# Autodesk Inventor assembly: one side of tower_MIR
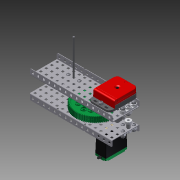
[picture p0: Inventor's stored thumbnail of the model, 180x180]
Saved by Autodesk Inventor 2014 SP1 (Build 180222100, 222)
## iProperties
Created: 2014-02-23
Part Number: one side of tower_MIR
Document SubType Name: Assembly
Designer: Ryan
Author: Ryan
## Documents named in this file (22)
- C:\Users\Ryan\Desktop\sw\toss up 4th robot\tower\one side of tower_MIR.iam
- C:\Users\Ryan\Desktop\sw\lib\Aperture VEX CAD Library\Metal\C Channel\5 x 15.ipt
- C:\Users\Ryan\Desktop\sw\lib\Aperture VEX CAD Library\Bearing Blocks\Bearing Block.ipt
- C:\Users\Ryan\Desktop\sw\lib\Aperture VEX CAD Library\Hardware\8-32\8-32 nylock.ipt
- C:\Users\Ryan\Desktop\sw\lib\Aperture VEX CAD Library\Hardware\8-32\8-32_.500.ipt
- C:\Users\Ryan\Desktop\sw\lib\Aperture VEX CAD Library\Spacers\thin\SPACER-0320-0125.ipt
- C:\Users\Ryan\Desktop\sw\lib\Aperture VEX CAD Library\Gears\High Strength Gears\HS-GEAR-12TOOTH.ipt
- C:\Users\Ryan\Desktop\sw\lib\Aperture VEX CAD Library\Hardware\8-32\8-32 nylock_MIR9.ipt
- C:\Users\Ryan\Desktop\sw\lib\Aperture VEX CAD Library\Spacers\thin\SPACER-0320-0500.ipt
- C:\Users\Ryan\Desktop\sw\lib\Aperture VEX CAD Library\Gears\High Strength Gears\Green HS 84.iam
- C:\Users\Ryan\Desktop\sw\lib\Aperture VEX CAD Library\Spacers\thin\SPACER-0320-0375.ipt
- C:\Users\Ryan\Desktop\sw\lib\Aperture VEX CAD Library\Hardware\Shaft Collar.ipt
- C:\Users\Ryan\Desktop\sw\lib\Aperture VEX CAD Library\Spacers\thin\SPACER-0320-0250.ipt
- C:\Users\Ryan\Desktop\sw\lib\Aperture VEX CAD Library\Standoffs\BEAM-1000.ipt
- C:\Users\Ryan\Desktop\sw\lib\Aperture VEX CAD Library\Hardware\8-32\8-32_.375.ipt
- C:\Users\Ryan\Desktop\sw\lib\Aperture VEX CAD Library\Standoffs\BEAM-0500.ipt
- C:\Users\Ryan\Desktop\sw\lib\Super Sonic Sparks VEX CAD Library\Motors & Sensors\2-Wire Motor 393-Without Wire.iam
- C:\Users\Ryan\Desktop\sw\lib\Aperture VEX CAD Library\Spacers\SPACER-0500-0250.ipt
- C:\Users\Ryan\Desktop\sw\lib\Aperture VEX CAD Library\Spacers\SPACER-0500-0625.ipt
- C:\Users\Ryan\Desktop\sw\lib\Aperture VEX CAD Library\Spacers\SPACER-0500-0125.ipt
- C:\Users\Ryan\Desktop\sw\lib\Aperture VEX CAD Library\Shaft\5.5 inch shaft.ipt
- C:\Users\Ryan\Desktop\sw\toss up 4th robot\tower\arm encoder.iam
## Components (66 placed, 21 different names)
1. 5 x 15:1 — Flush:4, Flush:2, Flush:1, Mate:3, Mate:2, Mate:5, Mate:4, Mate:11, Mate:13, Mate:30, Mate:31, Mate:44, Mate:43, Mate:122, Mate:121, Mate:47, Mate:55, Mate:56, Mate:57, Mate:62, Mate:73, Mate:77, Mate:82, Mate:81, Mate:80, Mate:104, Mate:105, Mate:106, Mate:127, Mate:126
2. 5 x 15:2 — Flush:4, Flush:2, Flush:1, Mate:123, Mate:35, Mate:23, Mate:26, Mate:36, Mate:66, Mate:124, Mate:70, Mate:69, Mate:79, Mate:93, Mate:96, Mate:117, Mate:120, Mate:132, Mate:140, Mate:132, Mate:133
3. Bearing Block:1 — Mate:3, Mate:2, Mate:9, Mate:8, Mate:7, Mate:6, Mate:5, Mate:4, Mate:61, Mate:125
4. 8-32 nylock:1 — Mate:9, Mate:8, Mate:12
5. 8-32 nylock:2 — Mate:7, Mate:6, Mate:10
6. 8-32_.500:1 — Mate:11, Mate:10, Flush:3
7. 8-32_.500:2 — Mate:12, Flush:3, Mate:95
8. SPACER-0320-0125:1 — Mate:13, Mate:16, Mate:15, Mate:33
9. HS-GEAR-12TOOTH:1 — Mate:16, Mate:15, Mate:145, Mate:144
10. Bearing Block:2 — Mate:123, Mate:35, Mate:23, Mate:20, Mate:19, Mate:18, Mate:17, Mate:28, Mate:27
11. 8-32 nylock:3 — Mate:20, Mate:19, Mate:22
12. 8-32 nylock_MIR9:1 — Mate:18, Mate:17, Mate:21
13. 8-32_.500:3 — Mate:26, Mate:21, Flush:5
14. 8-32_.500:4 — Mate:36, Mate:22, Flush:5
15. SPACER-0320-0500:1 — Mate:33, Mate:28, Mate:27, Mate:54
16. Green HS 84:1 [sub-assembly] — Mate:30, Mate:32, Mate:129
17. SPACER-0320-0125:2 — Mate:32, Mate:31, Mate:58
18. Bearing Block:3 — Mate:58, Mate:44, Mate:43, Mate:40, Mate:39, Mate:38, Mate:37
19. 8-32 nylock:4 — Mate:40, Mate:39, Mate:42
20. 8-32 nylock:5 — Mate:38, Mate:37, Mate:41
21. 8-32_.500:5 — Mate:122, Mate:41, Flush:6
22. 8-32_.500:6 — Mate:121, Mate:47, Mate:42, Flush:6
23. Bearing Block:4 — Mate:55, Mate:54, Mate:51, Mate:50, Mate:49, Mate:48, Flush:11
24. 8-32 nylock:6 — Mate:51, Mate:50, Mate:53
25. 8-32 nylock:7 — Mate:56, Mate:49, Mate:48, Mate:52
26. 8-32_.500:7 — Mate:57, Mate:52, Flush:7
27. 8-32_.500:8 — Mate:53, Flush:7
28. SPACER-0320-0125:3 — Mate:62, Mate:61, Mate:60, Mate:59, Mate:64
29. HS-GEAR-12TOOTH:2 — Mate:60, Mate:59
30. SPACER-0320-0375:1 — Mate:64, Mate:65, Mate:146
31. SPACER-0320-0125:4 — Mate:66, Mate:65, Mate:68, Mate:67
32. Shaft Collar:1 — Mate:146, Mate:68, Mate:67, Mate:94
33. SPACER-0320-0125:5 — Mate:124, Mate:70, Mate:69, Mate:72, Mate:78
34. SPACER-0320-0250:1 — Mate:73, Mate:72, Mate:75, Mate:74, Mate:76
35. BEAM-1000:1 — Mate:75, Mate:74
36. 8-32_.500:9 — Mate:77, Mate:76
37. 8-32_.375:1 — Mate:79, Mate:78
38. BEAM-0500:1 — Mate:82, Mate:81, Mate:80, Mate:103, Mate:136
39. Bearing Block:5 — Mate:95, Mate:94, Mate:93, Mate:90, Mate:89, Mate:88, Mate:87, Mate:131
40. 8-32 nylock:8 — Mate:90, Mate:89, Mate:92
41. 8-32 nylock:9 — Mate:88, Mate:87, Mate:91
42. 8-32_.500:10 — Mate:91, Flush:8
43. 8-32_.500:11 — Mate:96, Mate:92, Flush:8
44. Bearing Block:6 — Mate:104, Mate:103, Mate:100, Mate:99, Mate:98, Mate:97, Mate:108, Mate:107
45. 8-32 nylock:10 — Mate:100, Mate:99, Mate:102
46. 8-32 nylock:11 — Mate:105, Mate:98, Mate:97, Mate:101
47. 8-32_.500:12 — Mate:106, Mate:101, Flush:9
48. 8-32_.500:13 — Mate:102, Flush:9, Mate:119
49. 8-32_.500:14 — Mate:108, Mate:107
50. Bearing Block:7 — Mate:117, Mate:112, Mate:111, Mate:110, Mate:109, Mate:116, Mate:115
51. 8-32 nylock:12 — Mate:112, Mate:111, Mate:114
52. 8-32 nylock:13 — Mate:119, Mate:110, Mate:109, Mate:113
53. 8-32_.500:15 — Mate:113, Flush:10
54. 8-32_.500:16 — Mate:120, Mate:114, Flush:10
55. 8-32_.500:17 — Mate:116, Mate:115, Mate:141
56. 2-Wire Motor 393-Without Wire:1 [sub-assembly] — Mate:127, Mate:126, Mate:125
57. Shaft Collar:2 — Mate:129, Mate:131, Mate:130, Mate:134, Mate:133
58. SPACER-0500-0250:1 — Mate:131, Mate:130
59. SPACER-0500-0625:1 — Mate:134, Mate:133, Mate:132
60. SPACER-0500-0125:1 — Mate:136, Mate:137, Mate:135
61. SPACER-0500-0625:2 — Mate:137, Mate:135
62. SPACER-0500-0125:2 — Mate:141, Mate:139, Mate:138, Mate:143, Mate:142
63. SPACER-0500-0625:3 — Mate:140, Mate:139, Mate:138
64. 8-32 nylock:14 — Mate:143, Mate:142
65. 5.5 inch shaft:1 — Mate:145, Flush:11, Mate:144
66. arm encoder:1 [sub-assembly] — Mate:131, Mate:132, Mate:133
## Relationships (144: Mate 133, Flush 11)
- Flush:4 (50.8 mm): 5 x 15:1 ↔ 5 x 15:2
- Flush:2: 5 x 15:1 ↔ 5 x 15:2
- Flush:1: 5 x 15:1 ↔ 5 x 15:2
- Mate:3 (2.3114 mm): 5 x 15:1 ↔ Bearing Block:1
- Mate:2: 5 x 15:1 ↔ Bearing Block:1
- Mate:9: Bearing Block:1 ↔ 8-32 nylock:1
- Mate:8: Bearing Block:1 ↔ 8-32 nylock:1
- Mate:7: Bearing Block:1 ↔ 8-32 nylock:2
- Mate:6: Bearing Block:1 ↔ 8-32 nylock:2
- Mate:5 (53.1114 mm): 5 x 15:1 ↔ Bearing Block:1
- Mate:4 (-48.4886 mm): 5 x 15:1 ↔ Bearing Block:1
- Mate:11: 5 x 15:1 ↔ 8-32_.500:1
- Mate:10: 8-32 nylock:2 ↔ 8-32_.500:1
- Mate:12: 8-32 nylock:1 ↔ 8-32_.500:2
- Flush:3: 8-32_.500:1 ↔ 8-32_.500:2
- Mate:13: 5 x 15:1 ↔ SPACER-0320-0125:1
- Mate:16: SPACER-0320-0125:1 ↔ HS-GEAR-12TOOTH:1
- Mate:15: SPACER-0320-0125:1 ↔ HS-GEAR-12TOOTH:1
- Mate:123 (2.3114 mm): 5 x 15:2 ↔ Bearing Block:2
- Mate:35 (2.3114 mm): 5 x 15:2 ↔ Bearing Block:2
- Mate:23: 5 x 15:2 ↔ Bearing Block:2
- Mate:20: Bearing Block:2 ↔ 8-32 nylock:3
- Mate:19: Bearing Block:2 ↔ 8-32 nylock:3
- Mate:18: Bearing Block:2 ↔ 8-32 nylock_MIR9:1
- Mate:17: Bearing Block:2 ↔ 8-32 nylock_MIR9:1
- Mate:26: 5 x 15:2 ↔ 8-32_.500:3
- Mate:21: 8-32 nylock_MIR9:1 ↔ 8-32_.500:3
- Mate:36 (2.3114 mm): 5 x 15:2 ↔ 8-32_.500:4
- Mate:22: 8-32 nylock:3 ↔ 8-32_.500:4
- Flush:5: 8-32_.500:3 ↔ 8-32_.500:4
- Mate:33: SPACER-0320-0125:1 ↔ SPACER-0320-0500:1
- Mate:28: Bearing Block:2 ↔ SPACER-0320-0500:1
- Mate:27: Bearing Block:2 ↔ SPACER-0320-0500:1
- Mate:30 (3.175 mm): 5 x 15:1 ↔ Green HS 84:1
- Mate:32: Green HS 84:1 ↔ SPACER-0320-0125:2
- Mate:31: 5 x 15:1 ↔ SPACER-0320-0125:2
- Mate:58: SPACER-0320-0125:2 ↔ Bearing Block:3
- Mate:44 (2.3114 mm): 5 x 15:1 ↔ Bearing Block:3
- Mate:43: 5 x 15:1 ↔ Bearing Block:3
- Mate:40: Bearing Block:3 ↔ 8-32 nylock:4
- Mate:39: Bearing Block:3 ↔ 8-32 nylock:4
- Mate:38: Bearing Block:3 ↔ 8-32 nylock:5
- Mate:37: Bearing Block:3 ↔ 8-32 nylock:5
- Mate:122 (2.3114 mm): 5 x 15:1 ↔ 8-32_.500:5
- Mate:41: 8-32 nylock:5 ↔ 8-32_.500:5
- Mate:121 (2.3114 mm): 5 x 15:1 ↔ 8-32_.500:6
- Mate:47: 5 x 15:1 ↔ 8-32_.500:6
- Mate:42: 8-32 nylock:4 ↔ 8-32_.500:6
- Flush:6: 8-32_.500:5 ↔ 8-32_.500:6
- Mate:55: 5 x 15:1 ↔ Bearing Block:4
- Mate:54: SPACER-0320-0500:1 ↔ Bearing Block:4
- Mate:51: Bearing Block:4 ↔ 8-32 nylock:6
- Mate:50: Bearing Block:4 ↔ 8-32 nylock:6
- Mate:56 (2.3114 mm): 5 x 15:1 ↔ 8-32 nylock:7
- Mate:49: Bearing Block:4 ↔ 8-32 nylock:7
- Mate:48: Bearing Block:4 ↔ 8-32 nylock:7
- Mate:57: 5 x 15:1 ↔ 8-32_.500:7
- Mate:52: 8-32 nylock:7 ↔ 8-32_.500:7
- Mate:53: 8-32 nylock:6 ↔ 8-32_.500:8
- Flush:7: 8-32_.500:7 ↔ 8-32_.500:8
- Mate:62: 5 x 15:1 ↔ SPACER-0320-0125:3
- Mate:61: Bearing Block:1 ↔ SPACER-0320-0125:3
- Mate:60: SPACER-0320-0125:3 ↔ HS-GEAR-12TOOTH:2
- Mate:59: SPACER-0320-0125:3 ↔ HS-GEAR-12TOOTH:2
- Mate:64: SPACER-0320-0125:3 ↔ SPACER-0320-0375:1
- Mate:66: 5 x 15:2 ↔ SPACER-0320-0125:4
- Mate:65: SPACER-0320-0375:1 ↔ SPACER-0320-0125:4
- Mate:146: SPACER-0320-0375:1 ↔ Shaft Collar:1
- Mate:68: SPACER-0320-0125:4 ↔ Shaft Collar:1
- Mate:67: SPACER-0320-0125:4 ↔ Shaft Collar:1
- Mate:124 (2.3114 mm): 5 x 15:2 ↔ SPACER-0320-0125:5
- Mate:70 (2.3114 mm): 5 x 15:2 ↔ SPACER-0320-0125:5
- Mate:69: 5 x 15:2 ↔ SPACER-0320-0125:5
- Mate:73: 5 x 15:1 ↔ SPACER-0320-0250:1
- Mate:72: SPACER-0320-0125:5 ↔ SPACER-0320-0250:1
- Mate:75: SPACER-0320-0250:1 ↔ BEAM-1000:1
- Mate:74: SPACER-0320-0250:1 ↔ BEAM-1000:1
- Mate:77: 5 x 15:1 ↔ 8-32_.500:9
- Mate:76: SPACER-0320-0250:1 ↔ 8-32_.500:9
- Mate:79: 5 x 15:2 ↔ 8-32_.375:1
- Mate:78: SPACER-0320-0125:5 ↔ 8-32_.375:1
- Mate:82 (2.3114 mm): 5 x 15:1 ↔ BEAM-0500:1
- Mate:81 (2.3114 mm): 5 x 15:1 ↔ BEAM-0500:1
- Mate:80: 5 x 15:1 ↔ BEAM-0500:1
- Mate:95: 8-32_.500:2 ↔ Bearing Block:5
- Mate:94: Shaft Collar:1 ↔ Bearing Block:5
- Mate:93: 5 x 15:2 ↔ Bearing Block:5
- Mate:90: Bearing Block:5 ↔ 8-32 nylock:8
- Mate:89: Bearing Block:5 ↔ 8-32 nylock:8
- Mate:88: Bearing Block:5 ↔ 8-32 nylock:9
- Mate:87: Bearing Block:5 ↔ 8-32 nylock:9
- Mate:91: 8-32 nylock:9 ↔ 8-32_.500:10
- Mate:96: 5 x 15:2 ↔ 8-32_.500:11
- Mate:92: 8-32 nylock:8 ↔ 8-32_.500:11
- Flush:8: 8-32_.500:10 ↔ 8-32_.500:11
- Mate:104: 5 x 15:1 ↔ Bearing Block:6
- Mate:103: BEAM-0500:1 ↔ Bearing Block:6
- Mate:100: Bearing Block:6 ↔ 8-32 nylock:10
- Mate:99: Bearing Block:6 ↔ 8-32 nylock:10
- Mate:105 (2.3114 mm): 5 x 15:1 ↔ 8-32 nylock:11
- Mate:98: Bearing Block:6 ↔ 8-32 nylock:11
- Mate:97: Bearing Block:6 ↔ 8-32 nylock:11
- Mate:106: 5 x 15:1 ↔ 8-32_.500:12
- Mate:101: 8-32 nylock:11 ↔ 8-32_.500:12
- Mate:102: 8-32 nylock:10 ↔ 8-32_.500:13
- Flush:9: 8-32_.500:12 ↔ 8-32_.500:13
- Mate:108: Bearing Block:6 ↔ 8-32_.500:14
- Mate:107: Bearing Block:6 ↔ 8-32_.500:14
- Mate:117: 5 x 15:2 ↔ Bearing Block:7
- Mate:112: Bearing Block:7 ↔ 8-32 nylock:12
- Mate:111: Bearing Block:7 ↔ 8-32 nylock:12
- Mate:119: 8-32_.500:13 ↔ 8-32 nylock:13
- Mate:110: Bearing Block:7 ↔ 8-32 nylock:13
- Mate:109: Bearing Block:7 ↔ 8-32 nylock:13
- Mate:113: 8-32 nylock:13 ↔ 8-32_.500:15
- Mate:120: 5 x 15:2 ↔ 8-32_.500:16
- Mate:114: 8-32 nylock:12 ↔ 8-32_.500:16
- Flush:10: 8-32_.500:15 ↔ 8-32_.500:16
- Mate:116: Bearing Block:7 ↔ 8-32_.500:17
- Mate:115: Bearing Block:7 ↔ 8-32_.500:17
- Mate:127 (2.3114 mm): 5 x 15:1 ↔ 2-Wire Motor 393-Without Wire:1
- Mate:126: 5 x 15:1 ↔ 2-Wire Motor 393-Without Wire:1
- Mate:125: Bearing Block:1 ↔ 2-Wire Motor 393-Without Wire:1
- Mate:129: Green HS 84:1 ↔ Shaft Collar:2
- Mate:131: Shaft Collar:2 ↔ SPACER-0500-0250:1
- Mate:130: Shaft Collar:2 ↔ SPACER-0500-0250:1
- Mate:134: Shaft Collar:2 ↔ SPACER-0500-0625:1
- Mate:133: Shaft Collar:2 ↔ SPACER-0500-0625:1
- Mate:132: 5 x 15:2 ↔ SPACER-0500-0625:1
- Mate:136: BEAM-0500:1 ↔ SPACER-0500-0125:1
- Mate:137: SPACER-0500-0125:1 ↔ SPACER-0500-0625:2
- Mate:135: SPACER-0500-0125:1 ↔ SPACER-0500-0625:2
- Mate:141: 8-32_.500:17 ↔ SPACER-0500-0125:2
- Mate:140: 5 x 15:2 ↔ SPACER-0500-0625:3
- Mate:139: SPACER-0500-0125:2 ↔ SPACER-0500-0625:3
- Mate:138: SPACER-0500-0125:2 ↔ SPACER-0500-0625:3
- Mate:143: SPACER-0500-0125:2 ↔ 8-32 nylock:14
- Mate:142: SPACER-0500-0125:2 ↔ 8-32 nylock:14
- Mate:145: HS-GEAR-12TOOTH:1 ↔ 5.5 inch shaft:1
- Flush:11: Bearing Block:4 ↔ 5.5 inch shaft:1
- Mate:144: HS-GEAR-12TOOTH:1 ↔ 5.5 inch shaft:1
- Mate:131: Bearing Block:5 ↔ arm encoder:1
- Mate:132: 5 x 15:2 ↔ arm encoder:1
- Mate:133 (2.3114 mm): 5 x 15:2 ↔ arm encoder:1
## Named parameters: q = 2.3114 mm
